# Autodesk Inventor assembly: F.I.R.E.SAT Mk.2
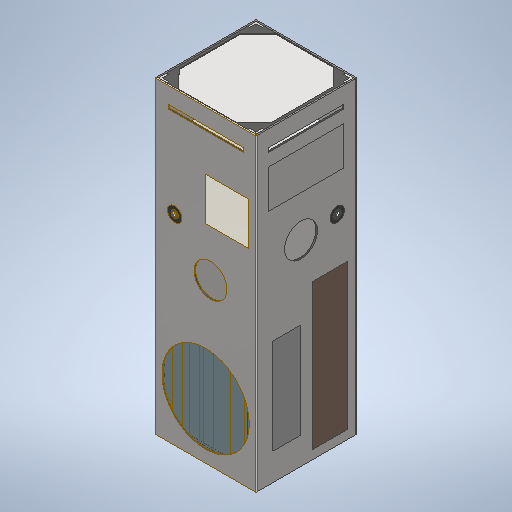
[picture p0: Inventor's stored thumbnail of the model, 512x512]
Saved by Autodesk Inventor 2025.3 (Build 293356000, 356)
## iProperties
Created: 2025-07-19
Part Number: F.I.R.E.SAT Mk.2
Document SubType Name: Assembly
Designer: kiran
Author: kiran
## Documents named in this file (14)
- C:\Users\kiran\Documents\F.I.R.E.SAT Project\Modal Analysis CAD.iam
- C:\Users\kiran\Documents\F.I.R.E.SAT Project\CAD Files\Mainframe Parts\Base Bracket.ipt
- C:\Users\kiran\Documents\F.I.R.E.SAT Project\CAD Files\Mainframe Parts\L-Bracket (Primary).ipt
- C:\Users\kiran\Documents\F.I.R.E.SAT Project\CAD Files\Mainframe Parts\Thermal Sensor Bracket.ipt
- C:\Users\kiran\Documents\F.I.R.E.SAT Project\CAD Files\Mainframe Parts\OBC Shelf.ipt
- C:\Users\kiran\Documents\F.I.R.E.SAT Project\CAD Files\Mainframe Parts\Universal Bracket.ipt
- C:\Users\kiran\Documents\F.I.R.E.SAT Project\CAD Files\Mainframe Parts\Support Rod.ipt
- C:\Users\kiran\Documents\F.I.R.E.SAT Project\CAD Files\Mainframe Parts\Support Rod - Thermal Sensor.ipt
- C:\Users\kiran\Documents\F.I.R.E.SAT Project\CAD Files\Mainframe Parts\Wall 1.ipt
- C:\Users\kiran\Documents\F.I.R.E.SAT Project\CAD Files\Mainframe Parts\Wall 3.ipt
- C:\Users\kiran\Documents\F.I.R.E.SAT Project\CAD Files\Mainframe Parts\Wall 4.ipt
- C:\Users\kiran\Documents\F.I.R.E.SAT Project\CAD Files\Mainframe Parts\Wall 2.ipt
- C:\Users\kiran\Documents\F.I.R.E.SAT Project\CAD Files\Mainframe Parts\Bottom Plate.ipt
- C:\Users\kiran\Documents\F.I.R.E.SAT Project\CAD Files\Mainframe Parts\Top Plate.ipt
## Components (22 placed, 13 different names)
1. Base Bracket:1 — Angle:1, Mate:38, Mate:39, Flush:2, Mate:40, Mate:41, Flush:3, Mate:42, Mate:43, Flush:4, Mate:44, Mate:45, Flush:5, Mate:68, Mate:69
2. Thermal Sensor Bracket:1 — Mate:47, Insert:17, Insert:18, Insert:19, Insert:20
3. OBC Shelf:1 — Insert:9, Insert:10, Insert:11, Insert:12, Mate:70, Mate:71, Mate:72
4. Support Rod:1 — Insert:9
5. Support Rod:2 — Insert:10
6. Support Rod:3 — Insert:11
7. Support Rod:4 — Insert:12
8. L-Bracket (Primary):1 — Mate:38, Mate:39, Flush:2, Mate:47, Flush:16, Mate:64
9. L-Bracket (Primary):2 — Mate:40, Mate:41, Flush:3, Flush:12, Mate:58, Flush:13, Mate:62, Flush:17, Mate:71
10. L-Bracket (Primary):3 — Mate:42, Mate:43, Flush:4, Flush:8, Flush:9, Mate:59, Flush:14, Mate:65, Mate:72, Mate:73
11. L-Bracket (Primary):4 — Mate:44, Mate:45, Flush:5, Mate:61, Flush:15, Mate:66, Mate:67, Mate:70
12. Universal Bracket:1 — Flush:8, Flush:9, Mate:73
13. Support Rod - Thermal Sensor:1 — Insert:17
14. Support Rod - Thermal Sensor:2 — Insert:18
15. Support Rod - Thermal Sensor:3 — Insert:20
16. Support Rod - Thermal Sensor:4 — Insert:19, Mate:68, Mate:69
17. Wall 3:1 — Flush:12, Mate:58, Flush:13, Mate:60, Mate:63
18. Wall 4:1 — Mate:59, Flush:14, Mate:60
19. Wall 1:1 — Mate:61, Flush:15, Flush:16, Flush:18, Flush:19
20. Wall 2:1 — Mate:62, Mate:63, Flush:17
21. Bottom Plate:1 — Mate:64, Flush:18, Mate:65
22. Top Plate:1 — Mate:66, Mate:67, Flush:19
## Relationships (48: Mate 25, Flush 14, Insert 8, Angle 1)
- Angle:1 (0 deg): Base Bracket:1
- Insert:9: OBC Shelf:1 ↔ Support Rod:1
- Insert:10: OBC Shelf:1 ↔ Support Rod:2
- Insert:11: OBC Shelf:1 ↔ Support Rod:3
- Insert:12: OBC Shelf:1 ↔ Support Rod:4
- Mate:38: Base Bracket:1 ↔ L-Bracket (Primary):1
- Mate:39: Base Bracket:1 ↔ L-Bracket (Primary):1
- Flush:2 (8 mm): Base Bracket:1 ↔ L-Bracket (Primary):1
- Mate:40: Base Bracket:1 ↔ L-Bracket (Primary):2
- Mate:41: Base Bracket:1 ↔ L-Bracket (Primary):2
- Flush:3 (-8 mm): Base Bracket:1 ↔ L-Bracket (Primary):2
- Mate:42: Base Bracket:1 ↔ L-Bracket (Primary):3
- Mate:43: Base Bracket:1 ↔ L-Bracket (Primary):3
- Flush:4 (-8 mm): Base Bracket:1 ↔ L-Bracket (Primary):3
- Mate:44: Base Bracket:1 ↔ L-Bracket (Primary):4
- Mate:45: Base Bracket:1 ↔ L-Bracket (Primary):4
- Flush:5 (8 mm): Base Bracket:1 ↔ L-Bracket (Primary):4
- Mate:47: Thermal Sensor Bracket:1 ↔ L-Bracket (Primary):1
- Flush:8: L-Bracket (Primary):3 ↔ Universal Bracket:1
- Flush:9: L-Bracket (Primary):3 ↔ Universal Bracket:1
- Insert:17: Thermal Sensor Bracket:1 ↔ Support Rod - Thermal Sensor:1
- Insert:18: Thermal Sensor Bracket:1 ↔ Support Rod - Thermal Sensor:2
- Insert:19: Thermal Sensor Bracket:1 ↔ Support Rod - Thermal Sensor:4
- Insert:20: Thermal Sensor Bracket:1 ↔ Support Rod - Thermal Sensor:3
- Flush:12: L-Bracket (Primary):2 ↔ Wall 3:1
- Mate:58: L-Bracket (Primary):2 ↔ Wall 3:1
- Flush:13 (-1.5 mm): L-Bracket (Primary):2 ↔ Wall 3:1
- Mate:59: L-Bracket (Primary):3 ↔ Wall 4:1
- Flush:14: L-Bracket (Primary):3 ↔ Wall 4:1
- Mate:60: Wall 3:1 ↔ Wall 4:1
- Mate:61: L-Bracket (Primary):4 ↔ Wall 1:1
- Flush:15: L-Bracket (Primary):4 ↔ Wall 1:1
- Flush:16 (1.5 mm): L-Bracket (Primary):1 ↔ Wall 1:1
- Mate:62: L-Bracket (Primary):2 ↔ Wall 2:1
- Mate:63: Wall 3:1 ↔ Wall 2:1
- Flush:17: L-Bracket (Primary):2 ↔ Wall 2:1
- Mate:64: L-Bracket (Primary):1 ↔ Bottom Plate:1
- Flush:18: Wall 1:1 ↔ Bottom Plate:1
- Mate:65: L-Bracket (Primary):3 ↔ Bottom Plate:1
- Mate:66: L-Bracket (Primary):4 ↔ Top Plate:1
- Mate:67: L-Bracket (Primary):4 ↔ Top Plate:1
- Flush:19: Wall 1:1 ↔ Top Plate:1
- Mate:68: Base Bracket:1 ↔ Support Rod - Thermal Sensor:4
- Mate:69: Base Bracket:1 ↔ Support Rod - Thermal Sensor:4
- Mate:70: OBC Shelf:1 ↔ L-Bracket (Primary):4
- Mate:71: OBC Shelf:1 ↔ L-Bracket (Primary):2
- Mate:72: OBC Shelf:1 ↔ L-Bracket (Primary):3
- Mate:73: L-Bracket (Primary):3 ↔ Universal Bracket:1
